# Autodesk Inventor assembly: assy
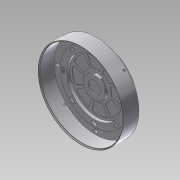
[picture p0: Inventor's stored thumbnail of the model, 180x180]
Saved by Autodesk Inventor 2019.3 (Build 233278000, 278)
## iProperties
Created: 2019-03-01
Part Number: assy
Document SubType Name: Assembly
Designer: WW
Author: WW
## Documents named in this file (7)
- D:\Dropbox\D4\assy.iam
- D:\Dropbox\D4\led_holster.ipt
- D:\Dropbox\D4\centre.ipt
- D:\Dropbox\D4\frosted_ring.ipt
- D:\Dropbox\D4\button_barrel.ipt
- D:\Dropbox\D4\wibble_ring.ipt
- D:\Dropbox\D4\bucket.ipt
## Components (6 placed, 6 different names)
1. led_holster:1 — Insert:2, Insert:5, Insert:7
2. centre:1 — Insert:7, Insert:8
3. frosted_ring:1 — Insert:2
4. button_barrel:1 — Insert:8
5. wibble_ring:1 — Insert:5, Angle:1, Insert:9
6. bucket:1 — Insert:9, Angle:2
## Relationships (7: Insert 5, Angle 2)
- Insert:2: led_holster:1 ↔ frosted_ring:1
- Insert:5: led_holster:1 ↔ wibble_ring:1
- Insert:7: led_holster:1 ↔ centre:1
- Insert:8: centre:1 ↔ button_barrel:1
- Angle:1 (0 deg): wibble_ring:1
- Insert:9: wibble_ring:1 ↔ bucket:1
- Angle:2 (0 deg): bucket:1
